# Autodesk Inventor assembly: Esper
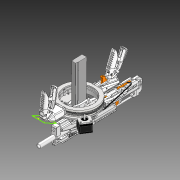
[picture p0: Inventor's stored thumbnail of the model, 180x180]
Saved by Autodesk Inventor 2020 (Build 240168000, 168)
## iProperties
Created: 2019-07-08
Part Number: Esper
Description: Alibre Inc.
Document SubType Name: Assembly
Designer: DDeGo
Sending System: Alibre
Preprocessor: ST-DEVELOPER v17
Title: export0
Revision Number: PRODUCT_VERSION_IDPRODUCT_VERSION_DESCR
## Documents named in this file (37)
- C:\Users\DDeGo\Documents\Drew\Projects\Nerf Aim Assist\ESPER\Esper.iam
- C:\Users\DDeGo\Documents\Drew\Projects\Nerf Aim Assist\ESPER\Barrel.ipt
- C:\Users\DDeGo\Documents\Drew\Projects\Nerf Aim Assist\ESPER\RamBase.ipt
- C:\Users\DDeGo\Documents\Drew\Projects\Nerf Aim Assist\ESPER\PlungerE.ipt
- C:\Users\DDeGo\Documents\Drew\Projects\Nerf Aim Assist\ESPER\PlungerTube.ipt
- C:\Users\DDeGo\Documents\Drew\Projects\Nerf Aim Assist\ESPER\Endcap.ipt
- C:\Users\DDeGo\Documents\Drew\Projects\Nerf Aim Assist\ESPER\Threaded Rod.ipt
- C:\Users\DDeGo\Documents\Drew\Projects\Nerf Aim Assist\ESPER\Dartjam.ipt
- C:\Users\DDeGo\Documents\Drew\Projects\Nerf Aim Assist\ESPER\Muzzle2.ipt
- C:\Users\DDeGo\Documents\Drew\Projects\Nerf Aim Assist\ESPER\Coupler.ipt
- C:\Users\DDeGo\Documents\Drew\Projects\Nerf Aim Assist\ESPER\Shockpad.ipt
- C:\Users\DDeGo\Documents\Drew\Projects\Nerf Aim Assist\ESPER\hexnut.ipt
- C:\Users\DDeGo\Documents\Drew\Projects\Nerf Aim Assist\ESPER\Cords.ipt
- C:\Users\DDeGo\Documents\Drew\Projects\Nerf Aim Assist\ESPER\RamCore.ipt
- C:\Users\DDeGo\Documents\Drew\Projects\Nerf Aim Assist\ESPER\frontpip.ipt
- C:\Users\DDeGo\Documents\Drew\Projects\Nerf Aim Assist\ESPER\pip.ipt
- C:\Users\DDeGo\Documents\Drew\Projects\Nerf Aim Assist\ESPER\BoltArm.ipt
- C:\Users\DDeGo\Documents\Drew\Projects\Nerf Aim Assist\ESPER\Foregrip6left.ipt
- C:\Users\DDeGo\Documents\Drew\Projects\Nerf Aim Assist\ESPER\Foregrip6right.ipt
- C:\Users\DDeGo\Documents\Drew\Projects\Nerf Aim Assist\ESPER\Tooth6.ipt
- C:\Users\DDeGo\Documents\Drew\Projects\Nerf Aim Assist\ESPER\ThreeQTube.ipt
- C:\Users\DDeGo\Documents\Drew\Projects\Nerf Aim Assist\ESPER\EBrake.ipt
- C:\Users\DDeGo\Documents\Drew\Projects\Nerf Aim Assist\ESPER\eVF1.ipt
- C:\Users\DDeGo\Documents\Drew\Projects\Nerf Aim Assist\ESPER\E-Pull2.ipt
- C:\Users\DDeGo\Documents\Drew\Projects\Nerf Aim Assist\ESPER\Spacer.ipt
- C:\Users\DDeGo\Documents\Drew\Projects\Nerf Aim Assist\ESPER\8inchTR.ipt
- C:\Users\DDeGo\Documents\Drew\Projects\Nerf Aim Assist\ESPER\TopSpacer.ipt
- C:\Users\DDeGo\Documents\Drew\Projects\Nerf Aim Assist\ESPER\EndLoop.ipt
- C:\Users\DDeGo\Documents\Drew\Projects\Nerf Aim Assist\ESPER\talon mag v1.ipt
- C:\Users\DDeGo\Documents\Drew\Projects\Nerf Aim Assist\ESPER\TopGrip.ipt
- C:\Users\DDeGo\Documents\Drew\Projects\Nerf Aim Assist\ESPER\Eforegrip2.ipt
- C:\Users\DDeGo\Documents\Drew\Projects\Nerf Aim Assist\ESPER\ETrigger.iam
- C:\Users\DDeGo\Documents\Drew\Projects\Nerf Aim Assist\Cad\127 x 146.05 x 12.7mm Printable Bearing Part 1.ipt
- C:\Users\DDeGo\Documents\Drew\Projects\Nerf Aim Assist\Cad\127 x 146.05 x 12.7mm Printable Bearing Part 2.ipt
- C:\Users\DDeGo\Documents\Drew\Projects\Nerf Aim Assist\Cad\MainMount.iam
- C:\Users\DDeGo\Documents\Drew\Projects\Nerf Aim Assist\Cad\BaseAssembly.iam
- C:\Users\DDeGo\Documents\Drew\Projects\Nerf Aim Assist\Cad\GearedUpper.ipt
## Components (39 placed, 39 different names)
1. NAUO_ID119 — Mate:2, Mate:3, Mate:15, Mate:28, Mate:38, Mate:61, Mate:62
2. NAUO_ID129 — Mate:29, Mate:31, Mate:32, Mate:37
3. NAUO_ID139 — Mate:30
4. NAUO_ID149 — Mate:22, Mate:23, Mate:31
5. NAUO_ID159 — Mate:34, Mate:35, Mate:36
6. NAUO_ID169 — Mate:9, Mate:14, Flush:1, Mate:26, Mate:43, Mate:64
7. NAUO_ID179 — Mate:3, Mate:5, Mate:7, Mate:21, Mate:38, Mate:57, Mate:59
8. NAUO_ID189 — Mate:7, Mate:8, Mate:9, Flush:1, Flush:2, Mate:57, Mate:63
9. NAUO_ID199 — Mate:8, Flush:2, Mate:25, Mate:42
10. NAUO_ID209 — Mate:14, Mate:15, Mate:23, Mate:45, Mate:52, Mate:53, Mate:65, Mate:66
11. NAUO_ID219 — Mate:33
12. NAUO_ID309
13. NAUO_ID319 — Mate:28, Mate:29, Mate:30, Mate:33, Mate:37
14. NAUO_ID329
15. NAUO_ID339
16. NAUO_ID369
17. NAUO_ID379
18. NAUO_ID389
19. NAUO_ID399
20. NAUO_ID409
21. NAUO_ID419
22. NAUO_ID429 — Mate:2, Mate:5
23. NAUO_ID439
24. NAUO_ID449 — Mate:20, Flush:3, Mate:22, Mate:32, Mate:59
25. NAUO_ID469
26. NAUO_ID489
27. NAUO_ID499
28. NAUO_ID509 — Mate:19, Mate:21, Flush:4
29. NAUO_ID519 — Mate:19, Mate:20, Flush:3
30. NAUO_ID609 — Mate:25, Mate:26, Mate:34, Mate:35, Mate:36, Flush:4, Mate:44
31. NAUO_ID629 — Mate:61, Mate:66, Angle:1
32. NAUO_ID659
33. NAUO_ID669
34. ETrigger:1 [sub-assembly] — Mate:42, Mate:43, Mate:44, Mate:45
35. 127 x 146.05 x 12.7mm Printable Bearing Part 1:1 — Mate:46, Flush:5, Mate:58, Mate:60
36. 127 x 146.05 x 12.7mm Printable Bearing Part 2:1 — Mate:46, Flush:5, Mate:50, Mate:51
37. MainMount:1 [sub-assembly] — Mate:50, Mate:51, Mate:52, Mate:53
38. BaseAssembly:1 [sub-assembly] — Mate:58, Mate:60
39. GearedUpper:1 — Mate:62, Mate:63, Mate:64, Mate:65, Angle:1
## Relationships (51: Mate 45, Flush 5, Angle 1)
- Mate:2: NAUO_ID119 ↔ NAUO_ID429
- Mate:3: NAUO_ID119 ↔ NAUO_ID179
- Mate:5: NAUO_ID179 ↔ NAUO_ID429
- Mate:7: NAUO_ID179 ↔ NAUO_ID189
- Mate:8: NAUO_ID189 ↔ NAUO_ID199
- Mate:9: NAUO_ID169 ↔ NAUO_ID189
- Mate:14: NAUO_ID169 ↔ NAUO_ID209
- Mate:15: NAUO_ID119 ↔ NAUO_ID209
- Flush:1: NAUO_ID169 ↔ NAUO_ID189
- Flush:2: NAUO_ID189 ↔ NAUO_ID199
- Mate:19: NAUO_ID509 ↔ NAUO_ID519
- Mate:20: NAUO_ID449 ↔ NAUO_ID519
- Flush:3: NAUO_ID449 ↔ NAUO_ID519
- Mate:21: NAUO_ID179 ↔ NAUO_ID509
- Mate:22: NAUO_ID149 ↔ NAUO_ID449
- Mate:23: NAUO_ID149 ↔ NAUO_ID209
- Mate:25: NAUO_ID199 ↔ NAUO_ID609
- Mate:26: NAUO_ID169 ↔ NAUO_ID609
- Mate:28: NAUO_ID119 ↔ NAUO_ID319
- Mate:29: NAUO_ID129 ↔ NAUO_ID319
- Mate:30: NAUO_ID139 ↔ NAUO_ID319
- Mate:31: NAUO_ID129 ↔ NAUO_ID149
- Mate:32: NAUO_ID129 ↔ NAUO_ID449
- Mate:33: NAUO_ID219 ↔ NAUO_ID319
- Mate:34: NAUO_ID159 ↔ NAUO_ID609
- Mate:35: NAUO_ID159 ↔ NAUO_ID609
- Mate:36: NAUO_ID159 ↔ NAUO_ID609
- Mate:37: NAUO_ID129 ↔ NAUO_ID319
- Mate:38: NAUO_ID119 ↔ NAUO_ID179
- Flush:4: NAUO_ID509 ↔ NAUO_ID609
- Mate:42: NAUO_ID199 ↔ ETrigger:1
- Mate:43: NAUO_ID169 ↔ ETrigger:1
- Mate:44: NAUO_ID609 ↔ ETrigger:1
- Mate:45: NAUO_ID209 ↔ ETrigger:1
- Mate:46: 127 x 146.05 x 12.7mm Printable Bearing Part 1:1 ↔ 127 x 146.05 x 12.7mm Printable Bearing Part 2:1
- Flush:5: 127 x 146.05 x 12.7mm Printable Bearing Part 1:1 ↔ 127 x 146.05 x 12.7mm Printable Bearing Part 2:1
- Mate:50: 127 x 146.05 x 12.7mm Printable Bearing Part 2:1 ↔ MainMount:1
- Mate:51: 127 x 146.05 x 12.7mm Printable Bearing Part 2:1 ↔ MainMount:1
- Mate:52: NAUO_ID209 ↔ MainMount:1
- Mate:53: NAUO_ID209 ↔ MainMount:1
- Mate:57: NAUO_ID179 ↔ NAUO_ID189
- Mate:58: 127 x 146.05 x 12.7mm Printable Bearing Part 1:1 ↔ BaseAssembly:1
- Mate:59: NAUO_ID179 ↔ NAUO_ID449
- Mate:60: 127 x 146.05 x 12.7mm Printable Bearing Part 1:1 ↔ BaseAssembly:1
- Mate:61: NAUO_ID119 ↔ NAUO_ID629
- Mate:62: NAUO_ID119 ↔ GearedUpper:1
- Mate:63: NAUO_ID189 ↔ GearedUpper:1
- Mate:64: NAUO_ID169 ↔ GearedUpper:1
- Mate:65: NAUO_ID209 ↔ GearedUpper:1
- Mate:66: NAUO_ID209 ↔ NAUO_ID629
- Angle:1 (180 deg): NAUO_ID629 ↔ GearedUpper:1
